# Autodesk Inventor assembly: plyta_dmd
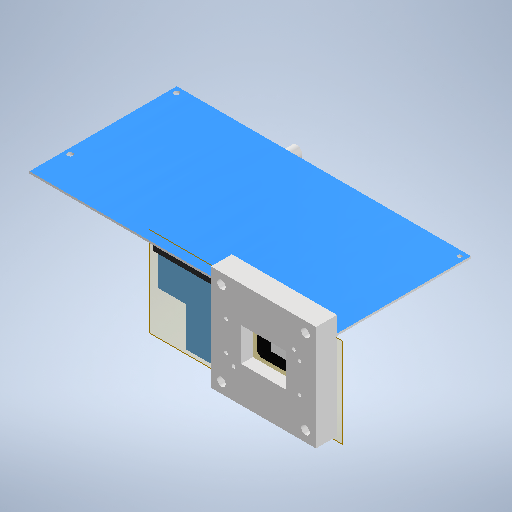
[picture p0: Inventor's stored thumbnail of the model, 512x512]
Saved by Autodesk Inventor 2025.1 (Build 291241000, 241)
## iProperties
Created: 2024-10-24
Part Number: plyta_dmd
Document SubType Name: Assembly
Designer: PC
Author: PC
## Documents named in this file (7)
- C:\Users\PC\Desktop\fotolito_czesci\nowe\plyta_dmd.iam
- C:\Users\PC\Desktop\fotolito_czesci\nowe\daughterboard.ipt
- C:\Users\PC\Desktop\fotolito_czesci\nowe\motherboard.ipt
- C:\Users\PC\Desktop\fotolito_czesci\nowe\podstawka.ipt
- C:\Users\PC\Desktop\fotolito_czesci\nowe\DLP.ipt
- C:\Users\PC\Desktop\fotolito_czesci\nowe\Część3.ipt
- C:\Users\PC\Desktop\fotolito_czesci\nowe\mocowanie_2000.ipt
## Components (6 placed, 6 different names)
1. daughterboard:1 — Zestawiające:1, Równoległe:1, Zestawiające:2, Zestawiające:3, Zestawiające:4, Zestawiające:5, Równoległe:3, Równoległe:4
2. motherboard:1 — Zestawiające:1, Równoległe:1, Zestawiające:2
3. podstawka:1 — Zestawiające:3, Zestawiające:4, Zestawiające:5, Zestawiające:6, Zestawiające:7, Zestawiające:8
4. DLP:1 — Zestawiające:6, Zestawiające:7, Zestawiające:8, Równoległe:2
5. Część3:1 — Równoległe:2
6. mocowanie_2000:1 — Równoległe:3, Równoległe:4
## Relationships (12: Mate 8, Flush 4)
- Zestawiające:1 [Mate] (1.6 mm): daughterboard:1 ↔ motherboard:1
- Równoległe:1 [Flush] (7 mm): daughterboard:1 ↔ motherboard:1
- Zestawiające:2 [Mate]: daughterboard:1 ↔ motherboard:1
- Zestawiające:3 [Mate]: daughterboard:1 ↔ podstawka:1
- Zestawiające:4 [Mate]: daughterboard:1 ↔ podstawka:1
- Zestawiające:5 [Mate]: daughterboard:1 ↔ podstawka:1
- Zestawiające:6 [Mate]: podstawka:1 ↔ DLP:1
- Zestawiające:7 [Mate]: podstawka:1 ↔ DLP:1
- Zestawiające:8 [Mate]: podstawka:1 ↔ DLP:1
- Równoległe:2 [Flush]: DLP:1 ↔ Część3:1
- Równoległe:3 [Flush]: daughterboard:1 ↔ mocowanie_2000:1
- Równoległe:4 [Flush]: daughterboard:1 ↔ mocowanie_2000:1
